# Autodesk Inventor assembly: CAM_T3
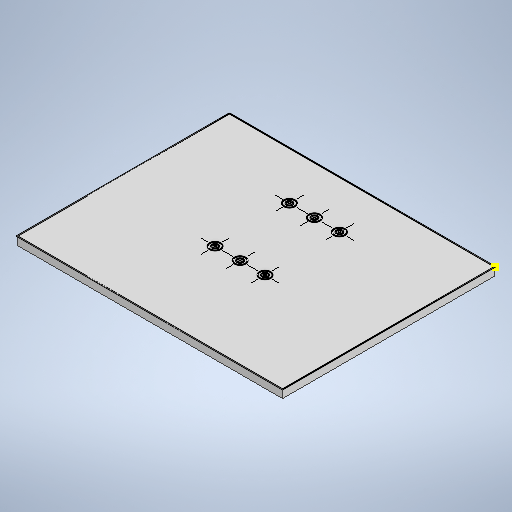
[picture p0: Inventor's stored thumbnail of the model, 512x512]
Saved by Autodesk Inventor 2025.2 (Build 292293000, 293)
## iProperties
Created: 2025-08-10
Part Number: CAM_T3
Document SubType Name: Assembly
Designer: User
Author: User
## Documents named in this file (2)
- C:\Users\User\Documents\The Maverick's Files\College 3-3\로보인 프로젝트\RHp_Humanoid_ver1\Part\Frame\Leg\Left Leg\CAM\CAM_T3.iam
- C:\Users\User\Documents\The Maverick's Files\College 3-3\로보인 프로젝트\RHp_Humanoid_ver1\Part\Frame\Leg\Left Leg\CAM\CAM_axis_6_bottom_frame(bottom).ipt
## Components (1 placed, 1 different names)
1. CAM_axis_6_bottom_frame(bottom):1 — Flush:1, Flush:2, Flush:3
## Relationships (3: Flush 3)
- Flush:1: CAM_axis_6_bottom_frame(bottom):1
- Flush:2: CAM_axis_6_bottom_frame(bottom):1
- Flush:3: CAM_axis_6_bottom_frame(bottom):1
